# Autodesk Inventor assembly: Kracken1
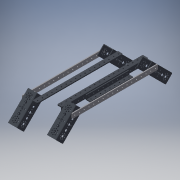
[picture p0: Inventor's stored thumbnail of the model, 180x180]
Saved by Autodesk Inventor 2016 (Build 200138000, 138)
## iProperties
Created: 2015-09-01
Part Number: Kracken1
Document SubType Name: Assembly
Designer: Tim
Author: Tim
## Documents named in this file (5)
- C:\Users\Tim\Documents\GitHub\phi_robotics\3d-models\FTC_Tetrix_KOP_Block_Party\Tim Bloot Designs\Kracken1.iam
- C:\Users\Tim\Documents\GitHub\phi_robotics\3d-models\FTC_Tetrix_KOP_Block_Party\Tetrix_Kit_FTC\Autodesk Inventor Files\tetrix_ANGLE - 288 MM.ipt
- C:\Users\Tim\Documents\GitHub\phi_robotics\3d-models\FTC_Tetrix_KOP_Block_Party\Tetrix_Kit_FTC\Autodesk Inventor Files\tetrix_FLAT BAR - 288 MM.ipt
- C:\Users\Tim\Documents\GitHub\phi_robotics\3d-models\FTC_Tetrix_KOP_Block_Party\Tetrix_Kit_FTC\Autodesk Inventor Files\tetrix_c_channel-2.ipt
- C:\Users\Tim\Documents\GitHub\phi_robotics\3d-models\FTC_Tetrix_KOP_Block_Party\Tetrix_Kit_FTC\Autodesk Inventor Files\tetrix_angle-144 MM.ipt
## Components (10 placed, 4 different names)
1. tetrix_ANGLE - 288 MM:1 — Rigid:1, Rigid:2, Rigid:10, Rigid:9
2. tetrix_ANGLE - 288 MM:2 — Rigid:5, Rigid:6, Rotational:1
3. tetrix_FLAT BAR - 288 MM:1 — Rigid:7, Rigid:8
4. tetrix_FLAT BAR - 288 MM:2 — Rigid:3, Rigid:4
5. tetrix_c_channel-2:1 — Rigid:1, Rigid:3
6. tetrix_c_channel-2:2 — Rigid:6, Rigid:7
7. tetrix_c_channel-2:3 — Rigid:5, Rigid:8
8. tetrix_c_channel-2:4 — Rigid:2, Rigid:4
9. tetrix_angle-144 MM:1 — Rigid:10, Rigid:9
10. tetrix_angle-144 MM:2 — Rotational:1
## Relationships (11: WeldJoint 10, RevoluteJoint 1)
- Rigid:1 [WeldJoint]: tetrix_ANGLE - 288 MM:1 ↔ tetrix_c_channel-2:1
- Rigid:2 [WeldJoint]: tetrix_ANGLE - 288 MM:1 ↔ tetrix_c_channel-2:4
- Rigid:3 [WeldJoint]: tetrix_FLAT BAR - 288 MM:2 ↔ tetrix_c_channel-2:1
- Rigid:4 [WeldJoint]: tetrix_FLAT BAR - 288 MM:2 ↔ tetrix_c_channel-2:4
- Rigid:5 [WeldJoint]: tetrix_ANGLE - 288 MM:2 ↔ tetrix_c_channel-2:3
- Rigid:6 [WeldJoint]: tetrix_ANGLE - 288 MM:2 ↔ tetrix_c_channel-2:2
- Rigid:7 [WeldJoint]: tetrix_FLAT BAR - 288 MM:1 ↔ tetrix_c_channel-2:2
- Rigid:8 [WeldJoint]: tetrix_FLAT BAR - 288 MM:1 ↔ tetrix_c_channel-2:3
- Rotational:1 [RevoluteJoint]: tetrix_ANGLE - 288 MM:2 ↔ tetrix_angle-144 MM:2
- Rigid:10 [WeldJoint]: tetrix_ANGLE - 288 MM:1 ↔ tetrix_angle-144 MM:1
- Rigid:9 [WeldJoint]: tetrix_ANGLE - 288 MM:1 ↔ tetrix_angle-144 MM:1
